# Autodesk Inventor assembly: X_Carriage_Cyclops_Ir
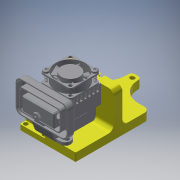
[picture p0: Inventor's stored thumbnail of the model, 180x180]
Saved by Autodesk Inventor 2019 (Build 230136000, 136)
## iProperties
Created: 2019-07-20
Part Number: X_Carriage_Cyclops_Ir
Material: Generisch
Document SubType Name: Assembly
Designer: marc
Author: marc
## Documents named in this file (4)
- C:\Users\marc\Google Drive\Projekte\3D Drucker\brezzlicator\1. Printed Parts\3. Modified by marc\inventor\X_Carriage_Cyclops_Ir.iam
- C:\Users\marc\Downloads\uploads_c5_d5_d4_97_4f_Cyclops.iam
- C:\Users\marc\Google Drive\Projekte\3D Drucker\brezzlicator\1. Printed Parts\3. Modified by marc\inventor\Extruder Mount cyclops mit ir probe.ipt
- C:\Users\marc\Google Drive\Projekte\3D Drucker\brezzlicator\1. Printed Parts\3. Modified by marc\inventor\duct_v6.ipt
## Components (3 placed, 3 different names)
1. uploads_c5_d5_d4_97_4f_Cyclops:1 [sub-assembly] — Starr:1, Drehbar:1
2. Extruder Mount cyclops mit ir probe:1 — Starr:1, Drehbar:1, Starr:2
3. duct_v6:1 — Starr:2
## Relationships (3: WeldJoint 2, RevoluteJoint 1)
- Starr:1 [WeldJoint]: uploads_c5_d5_d4_97_4f_Cyclops:1 ↔ Extruder Mount cyclops mit ir probe:1
- Drehbar:1 [RevoluteJoint]: uploads_c5_d5_d4_97_4f_Cyclops:1 ↔ Extruder Mount cyclops mit ir probe:1
- Starr:2 [WeldJoint]: Extruder Mount cyclops mit ir probe:1 ↔ duct_v6:1
